# Autodesk Inventor assembly: FrontWheelAssembly
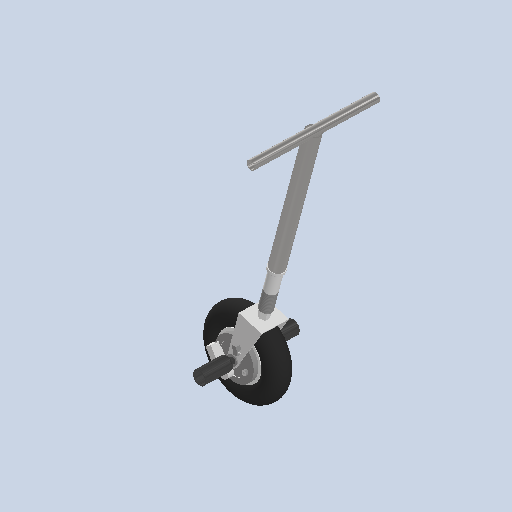
[picture p0: Inventor's stored thumbnail of the model, 512x512]
Saved by Autodesk Inventor 2022.2 (Build 262287010, 287A)
## iProperties
_SolveAssemblyDoc: Frame Generator Solve Assembly
_Version: 15.0.0
Created: 2022-04-08
Part Number: FrontWheelAssembly
Document SubType Name: Assembly
Designer: Finn Oriwohl
Author: Finn Oriwohl
## Documents named in this file (7)
- C:\Users\Finn Oriwohl\Documents\htx\1g g\BeerCart-CAD-Inventor\Workspaces\Workspace\FrontWheelAssembly.iam
- C:\Users\Finn Oriwohl\Documents\htx\1g g\BeerCart-CAD-Inventor\Workspaces\Workspace\frontwheelFork.ipt
- C:\Users\Finn Oriwohl\Documents\htx\1g g\BeerCart-CAD-Inventor\Workspaces\Workspace\FreeBackWheel.ipt
- C:\Users\Finn Oriwohl\Documents\htx\1g g\BeerCart-CAD-Inventor\Workspaces\Workspace\pegsFront wheel.ipt
- C:\Users\Finn Oriwohl\Documents\htx\1g g\BeerCart-CAD-Inventor\Workspaces\Workspace\headset bearing.ipt
- C:\Users\Finn Oriwohl\Documents\htx\1g g\BeerCart-CAD-Inventor\Workspaces\Workspace\FrontWheelAssembly\Frame\Frame 1649413593822.iam
- C:\Users\Finn Oriwohl\Documents\htx\1g g\BeerCart-CAD-Inventor\Workspaces\Workspace\FrontWheelHandle.ipt
## Components (7 placed, 6 different names)
1. headset bearing:1 — Insert:4, Mate:1, Flush:1
2. frontwheelFork:1 — Mate:1, Flush:1, Mate:2, Angle:1
3. FreeBackWheel:1
4. pegsFront wheel:1
5. pegsFront wheel:2
6. Frame 1649413593822:1 [sub-assembly] — Insert:4
7. FrontWheelHandle:1 — Flush:2, Flush:3
## Relationships (11: Insert 4, Mate 3, Flush 3, Angle 1)
- [Insert] (-5 mm): frontwheelFork:1 ↔ FreeBackWheel:1
- [Insert]: frontwheelFork:1 ↔ pegsFront wheel:1
- [Insert]: frontwheelFork:1 ↔ pegsFront wheel:2
- Insert:4: headset bearing:1 ↔ Frame 1649413593822:1
- Mate:1: headset bearing:1 ↔ frontwheelFork:1
- Flush:1 (35 mm): headset bearing:1 ↔ frontwheelFork:1
- Mate:2: frontwheelFork:1
- Mate:3
- Angle:1 (90 deg): frontwheelFork:1
- Flush:2: FrontWheelHandle:1
- Flush:3: FrontWheelHandle:1
